# Autodesk Inventor assembly: mecanumL
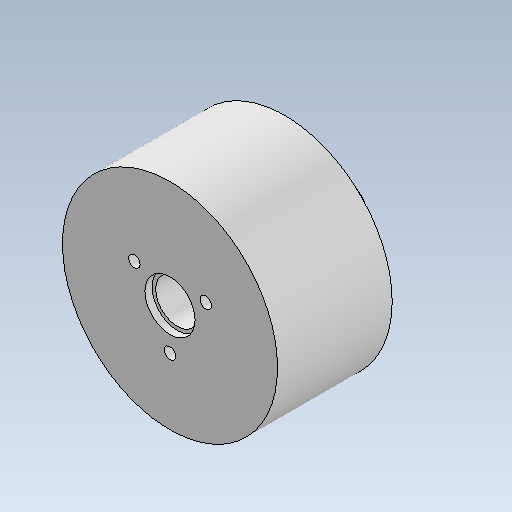
[picture p0: Inventor's stored thumbnail of the model, 512x512]
Saved by Autodesk Inventor 2026.1 (Build 301233020, 233B)
## iProperties
Created: 2026-10-09
Part Number: mecanumL
Document SubType Name: Assembly
Designer: ug_nd
Author: ug_nd
## Documents named in this file (3)
- C:\Users\ug_nd\git_local\3wd_mecanums\cad\common_parts\mecanumL.iam
- C:\Users\ug_nd\git_local\3wd_mecanums\cad\common_parts\mecanumL.ipt
- C:\Users\ug_nd\git_local\3wd_mecanums\cad\common_parts\mecanum_hub.ipt
## Components (2 placed, 2 different names)
1. mecanumL:1 — メイト:1, メイト:2, メイト:3
2. mecanum_hub:1 — メイト:1, メイト:2, メイト:3
## Relationships (3: Mate 3)
- メイト:1 [Mate]: mecanumL:1 ↔ mecanum_hub:1
- メイト:2 [Mate]: mecanumL:1 ↔ mecanum_hub:1
- メイト:3 [Mate]: mecanumL:1 ↔ mecanum_hub:1
